# Autodesk Inventor assembly: POM_T5_09
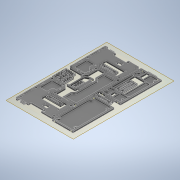
[picture p0: Inventor's stored thumbnail of the model, 180x180]
Saved by Autodesk Inventor 2022 (Build 260153000, 153)
## iProperties
Created: 2022-09-28
Part Number: POM_T5_09
Document SubType Name: Assembly
Designer: Masato
Author: Masato
## Documents named in this file (10)
- C:\Users\ヨコオリク\Documents\CITBrains\SUSTAINA-OP\Cam\POM_T5\POM_T5_09.iam
- C:\Users\ヨコオリク\Documents\CITBrains\SUSTAINA-OP\Cam\DisposableBoard.ipt
- C:\Users\ヨコオリク\Documents\CITBrains\SUSTAINA-OP\UpperBody\Cockpit\Cockpit_back_frame.ipt
- C:\Users\ヨコオリク\Documents\CITBrains\SUSTAINA-OP\UpperBody\Cockpit\Cockpit_battery_back_door.ipt
- C:\Users\ヨコオリク\Documents\CITBrains\SUSTAINA-OP\UpperBody\Cockpit\Cockpit_carrier_board_frame.ipt
- C:\Users\ヨコオリク\Documents\CITBrains\SUSTAINA-OP\UpperBody\Cockpit\Cockpit_front_frame.ipt
- C:\Users\ヨコオリク\Documents\CITBrains\SUSTAINA-OP\UpperBody\Cockpit\Cockpit_side_frame.ipt
- C:\Users\ヨコオリク\Documents\CITBrains\SUSTAINA-OP\UpperBody\Cockpit\Cockpit_side_frame_MIR.ipt
- C:\Users\ヨコオリク\Documents\CITBrains\SUSTAINA-OP\OptionParts\DrillingJigs\Head_neck_diagonal_Jig_back.ipt
- C:\Users\ヨコオリク\Documents\CITBrains\SUSTAINA-OP\OptionParts\DrillingJigs\Head_neck_diagonal_Jig_side.ipt
## Components (17 placed, 9 different names)
1. DisposableBoard:1 — フラッシュ:1, フラッシュ:2, フラッシュ:3, フラッシュ:4, フラッシュ:5, フラッシュ:6, フラッシュ:14, フラッシュ:15
2. Cockpit_back_frame:1 — メイト:5, フラッシュ:12, フラッシュ:13, メイト:18, メイト:19
3. Cockpit_battery_back_door:1 — メイト:3, メイト:12, フラッシュ:10, メイト:13, メイト:15, メイト:24
4. Cockpit_front_frame:1 — メイト:1, フラッシュ:11, メイト:14, フラッシュ:13, メイト:25
5. Cockpit_side_frame:1 — メイト:7, フラッシュ:5, フラッシュ:6, フラッシュ:9, メイト:12, フラッシュ:10, フラッシュ:11, メイト:14, 正接:1, メイト:20, メイト:27, メイト:28
6. Cockpit_side_frame_MIR:1 — メイト:11, フラッシュ:9, メイト:13, フラッシュ:12, メイト:30, メイト:31
7. Cockpit_carrier_board_frame:2 — メイト:10, メイト:15, 正接:1, メイト:33, メイト:34
8. Head_neck_diagonal_Jig_side:4 — メイト:21, フラッシュ:15, メイト:22
9. Head_neck_diagonal_Jig_back:3 — メイト:23, メイト:24, メイト:25
10. Head_neck_diagonal_Jig_back:4 — メイト:26, メイト:27, メイト:28
11. Head_neck_diagonal_Jig_back:5 — メイト:29, メイト:30, メイト:31
12. Head_neck_diagonal_Jig_side:5 — メイト:32, メイト:33, メイト:34
13. Head_neck_diagonal_Jig_back:1 — メイト:16, メイト:18, メイト:19
14. Head_neck_diagonal_Jig_back:2
15. Head_neck_diagonal_Jig_side:1 — メイト:17, メイト:20, フラッシュ:14, メイト:22
16. Head_neck_diagonal_Jig_side:2
17. Head_neck_diagonal_Jig_side:3
## Component patterns: (2 elements, first: Head_neck_diagonal_Jig_back:1), (3 elements, first: Head_neck_diagonal_Jig_side:1)
## Relationships (43: Mate 29, Flush 13, Tangent 1)
- フラッシュ:1 [Flush]: DisposableBoard:1
- フラッシュ:2 [Flush]: DisposableBoard:1
- フラッシュ:3 [Flush]: DisposableBoard:1
- フラッシュ:4 [Flush]: DisposableBoard:1
- メイト:1 [Mate]: Cockpit_front_frame:1
- メイト:3 [Mate]: Cockpit_battery_back_door:1
- メイト:5 [Mate]: Cockpit_back_frame:1
- メイト:7 [Mate]: Cockpit_side_frame:1
- メイト:10 [Mate]: Cockpit_carrier_board_frame:2
- メイト:11 [Mate]: Cockpit_side_frame_MIR:1
- フラッシュ:5 [Flush] (-2 mm): DisposableBoard:1 ↔ Cockpit_side_frame:1
- フラッシュ:6 [Flush] (2 mm): DisposableBoard:1 ↔ Cockpit_side_frame:1
- フラッシュ:9 [Flush]: Cockpit_side_frame:1 ↔ Cockpit_side_frame_MIR:1
- メイト:12 [Mate] (2.1 mm): Cockpit_battery_back_door:1 ↔ Cockpit_side_frame:1
- フラッシュ:10 [Flush]: Cockpit_battery_back_door:1 ↔ Cockpit_side_frame:1
- メイト:13 [Mate] (2.1 mm): Cockpit_battery_back_door:1 ↔ Cockpit_side_frame_MIR:1
- フラッシュ:11 [Flush]: Cockpit_front_frame:1 ↔ Cockpit_side_frame:1
- フラッシュ:12 [Flush]: Cockpit_back_frame:1 ↔ Cockpit_side_frame_MIR:1
- メイト:14 [Mate] (2.1 mm): Cockpit_front_frame:1 ↔ Cockpit_side_frame:1
- フラッシュ:13 [Flush]: Cockpit_back_frame:1 ↔ Cockpit_front_frame:1
- メイト:15 [Mate] (2.1 mm): Cockpit_battery_back_door:1 ↔ Cockpit_carrier_board_frame:2
- 正接:1 [Tangent] (2.1 mm): Cockpit_side_frame:1 ↔ Cockpit_carrier_board_frame:2
- メイト:16 [Mate]: Head_neck_diagonal_Jig_back:1
- メイト:17 [Mate]: Head_neck_diagonal_Jig_side:1
- メイト:18 [Mate] (2.1 mm): Cockpit_back_frame:1 ↔ Head_neck_diagonal_Jig_back:1
- メイト:19 [Mate] (2.1 mm): Cockpit_back_frame:1 ↔ Head_neck_diagonal_Jig_back:1
- メイト:20 [Mate] (2.1 mm): Cockpit_side_frame:1 ↔ Head_neck_diagonal_Jig_side:1
- フラッシュ:14 [Flush] (2 mm): DisposableBoard:1 ↔ Head_neck_diagonal_Jig_side:1
- メイト:21 [Mate]: Head_neck_diagonal_Jig_side:4
- フラッシュ:15 [Flush] (2 mm): DisposableBoard:1 ↔ Head_neck_diagonal_Jig_side:4
- メイト:22 [Mate] (2.1 mm): Head_neck_diagonal_Jig_side:4 ↔ Head_neck_diagonal_Jig_side:1
- メイト:23 [Mate]: Head_neck_diagonal_Jig_back:3
- メイト:24 [Mate] (2.1 mm): Cockpit_battery_back_door:1 ↔ Head_neck_diagonal_Jig_back:3
- メイト:25 [Mate] (2.1 mm): Cockpit_front_frame:1 ↔ Head_neck_diagonal_Jig_back:3
- メイト:26 [Mate]: Head_neck_diagonal_Jig_back:4
- メイト:27 [Mate] (2.1 mm): Cockpit_side_frame:1 ↔ Head_neck_diagonal_Jig_back:4
- メイト:28 [Mate] (2.1 mm): Cockpit_side_frame:1 ↔ Head_neck_diagonal_Jig_back:4
- メイト:29 [Mate]: Head_neck_diagonal_Jig_back:5
- メイト:30 [Mate] (2.1 mm): Cockpit_side_frame_MIR:1 ↔ Head_neck_diagonal_Jig_back:5
- メイト:31 [Mate] (2.1 mm): Cockpit_side_frame_MIR:1 ↔ Head_neck_diagonal_Jig_back:5
- メイト:32 [Mate]: Head_neck_diagonal_Jig_side:5
- メイト:33 [Mate] (2.1 mm): Cockpit_carrier_board_frame:2 ↔ Head_neck_diagonal_Jig_side:5
- メイト:34 [Mate] (2.1 mm): Cockpit_carrier_board_frame:2 ↔ Head_neck_diagonal_Jig_side:5
